# Autodesk Inventor assembly: glass
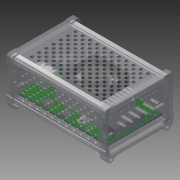
[picture p0: Inventor's stored thumbnail of the model, 180x180]
Saved by Autodesk Inventor 2013 SP1 (Build 170176100, 176)
## iProperties
Created: 2019-01-15
Part Number: glass
Document SubType Name: Assembly
Designer: jhcjhguw
Author: jhcjhguw
## Documents named in this file (8)
- D:\InventorProject\Artix200_case\glass\glass.iam
- D:\InventorProject\Artix200_case\glass\bottom.ipt
- D:\InventorProject\Artix200_case\glass\profile.ipt
- D:\InventorProject\Artix200_case\glass\side.ipt
- D:\InventorProject\Artix200_case\glass\top.ipt
- D:\InventorProject\Artix200_case\glass\front.ipt
- D:\InventorProject\Artix200_case\plast_board_assembled.iam
- D:\InventorProject\Artix200_case\glass\back.ipt
## Components (11 placed, 7 different names)
1. bottom:1 — Совмещение:1, Заподлицо:1, Совмещение:2, Совмещение:3, Заподлицо:2, Совмещение:4, Совмещение:18, Совмещение:22
2. profile:1 — Совмещение:9, Заподлицо:5, Совмещение:10, Совмещение:24
3. profile:2 — Совмещение:11, Заподлицо:6, Совмещение:12, Совмещение:13, Заподлицо:7, Совмещение:14
4. profile:3 — Совмещение:3, Заподлицо:2, Совмещение:4, Совмещение:5, Заподлицо:3, Совмещение:6
5. profile:4 — Совмещение:1, Заподлицо:1, Совмещение:2, Совмещение:7, Заподлицо:4, Совмещение:8, Совмещение:20
6. side:1 — Совмещение:5, Заподлицо:3, Совмещение:6, Совмещение:11, Заподлицо:6, Совмещение:12
7. side:2 — Совмещение:7, Заподлицо:4, Совмещение:8, Совмещение:9, Заподлицо:5, Совмещение:10, Совмещение:19, Совмещение:21, Совмещение:26
8. top:1 — Совмещение:13, Заподлицо:7, Совмещение:14, Совмещение:25
9. plast_board_assembled:1 [sub-assembly] — Совмещение:18, Совмещение:19, Совмещение:23
10. front:1 — Совмещение:20, Совмещение:21, Совмещение:22, Совмещение:23
11. back:1 — Совмещение:24, Совмещение:25, Совмещение:26
## Relationships (30: Mate 23, Flush 7)
- Совмещение:1 [Mate]: bottom:1 ↔ profile:4
- Заподлицо:1 [Flush]: bottom:1 ↔ profile:4
- Совмещение:2 [Mate]: bottom:1 ↔ profile:4
- Совмещение:3 [Mate]: bottom:1 ↔ profile:3
- Заподлицо:2 [Flush]: bottom:1 ↔ profile:3
- Совмещение:4 [Mate]: bottom:1 ↔ profile:3
- Совмещение:5 [Mate]: profile:3 ↔ side:1
- Заподлицо:3 [Flush]: profile:3 ↔ side:1
- Совмещение:6 [Mate]: profile:3 ↔ side:1
- Совмещение:7 [Mate]: profile:4 ↔ side:2
- Заподлицо:4 [Flush]: profile:4 ↔ side:2
- Совмещение:8 [Mate]: profile:4 ↔ side:2
- Совмещение:9 [Mate]: profile:1 ↔ side:2
- Заподлицо:5 [Flush]: profile:1 ↔ side:2
- Совмещение:10 [Mate]: profile:1 ↔ side:2
- Совмещение:11 [Mate]: profile:2 ↔ side:1
- Заподлицо:6 [Flush]: profile:2 ↔ side:1
- Совмещение:12 [Mate]: profile:2 ↔ side:1
- Совмещение:13 [Mate]: profile:2 ↔ top:1
- Заподлицо:7 [Flush]: profile:2 ↔ top:1
- Совмещение:14 [Mate]: profile:2 ↔ top:1
- Совмещение:18 [Mate] (5 mm): bottom:1 ↔ plast_board_assembled:1
- Совмещение:19 [Mate] (2.6 mm): side:2 ↔ plast_board_assembled:1
- Совмещение:20 [Mate]: profile:4 ↔ front:1
- Совмещение:21 [Mate]: side:2 ↔ front:1
- Совмещение:22 [Mate]: bottom:1 ↔ front:1
- Совмещение:23 [Mate]: plast_board_assembled:1 ↔ front:1
- Совмещение:24 [Mate]: profile:1 ↔ back:1
- Совмещение:25 [Mate]: top:1 ↔ back:1
- Совмещение:26 [Mate]: side:2 ↔ back:1
